# Autodesk Inventor assembly: 042-P(F,D-166-3)
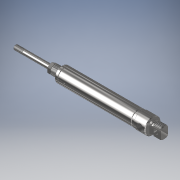
[picture p0: Inventor's stored thumbnail of the model, 180x180]
Saved by Autodesk Inventor 2017 (Build 210142000, 142)
## iProperties
Category: PARTsolutions
Company: BIMBA
Created: 2016-10-01
Part Number: 042-P(F,D-166-3)
Catalog Web Link: www.cadenas.de
Description: Original Line Standard Air Cylinders-
Vendor: BIMBA
Document SubType Name: Assembly
Designer: psAdmin
Manufacturer: BIMBA
PSOL_IDENT_0: {$CADENAS_DATA\23d-libs\bimba\bimba\bimba_imperial\bimba_full_line\original_line_cylinders\standard_
PSOL_IDENT_1: air_cylinders\standard_air_cylinder_asmtab.prj},321 {VTYP=3D},{STYP=ASSTAB},{NB=042-P(F,D-166-3)},{L
PSOL_IDENT_2: INA=042-P},{NN=Original Line Standard Air Cylinders},{DATE=22.09.2016 13:52:24},{GEOMDATE=11.07.2016
PSOL_IDENT_3: 10:37:18},{VERSION=},{LINEID=50},{LINESUBID=-1},{WBVAR=STROKE,ACTING,MNT,DER,NR,BM,CO,OO,VO,M,EE,EE
PSOL_IDENT_4: L,K,Q,Y,G,T,B,H,SER,SR,NT,W,HL,STPT1,STPT2,STPT3,STPT4,MB,PB,PRC,TB,MN}  {NB=042-P(F,D-166-3)},{LINA=
PSOL_IDENT_5: 042-P},{KT=DUMMY},{PN=042-P},{PNC=042-P(F,D-166-3)},{PNA=(D-166-3)},{DASH=-},{BORE1=0.75000000},{BOR
PSOL_IDENT_6: E=3/4\" (04)},{BOREPN=04},{STROKE=2.000},{STROKEALG=[0.011:50/0.001]},{STROKE1=2.000},{ACTING=},{ACT
PSOL_IDENT_7: INGALG= '' , 'Single Acting (SA)' , 'R' , 'Reverse Single Acting (SA)' , 'D' , 'Double Acting (SA)'
PSOL_IDENT_8: },{ACTINGPN=},{MNT=P},{MNTALG= '' , 'Front Nose Mounting (SA)' , 'P' , 'Rear Pivot Mounting (SA)' , '
PSOL_IDENT_9: BF' , 'Front Block Mounting (SA)' , 'BR' , 'Rear Block Mounting for Vertical Positioning (SA)' , 'BF
PSOL_IDENT_10: T' , 'Front Block Trunnion Mounting (SA)' , 'BRT' , 'Rear Block Trunnion Mounting (SA)' , 'A' , 'Dou
PSOL_IDENT_11: ble End Mounting with Brackets and Adjustable Stroke (SA)' , 'AP' , 'Rear Pivot Mounting with Adjust
PSOL_IDENT_12: able Stroke (SA)' },{TYPE=},{MNTPN=P},{DER=},{DERALG= '' , 'N/A' },{NR=},{NRALG= '' , 'Round (Standa
PSOL_IDENT_13: rd)' , 'NR' , 'Non-rotating - Hexagon Rod' },{NRPN=},{BM=},{BMALG= '' , 'N/A' },{BMPN=},{CO=},{COALG=
PSOL_IDENT_14: '' , 'N/A' },{OO=},{OOALG= '', 'N/A' },{OOPN=},{VO=Z},{VOALG= 'Z' , 'N/A' },{VOPN=},{OOVOPN=},{M=},
PSOL_IDENT_15: {MALG= '', 'Without Magnet', 'M', 'With Magnet' },{EE=},{EEL=0.000},{EEMAX=48.0000},{EEALG= '', 'Wit
PSOL_IDENT_16: hout Extra Extension', 'EE', 'With Extra Extension' },{EELALG=0},{EEPN=},{EEPN1=0.000},{K=},{KALG= ''
PSOL_IDENT_17: , 'Standard' , 'K' , 'Ports Rotated 90deg K' },{KPN=},{Q=},{QALG= '' , 'N/A' },{QPN=},{Y=},{YALG= ''
PSOL_IDENT_18: , 'Without Pivot Bushing' , 'Y' , 'With Pivot Bushing' },{YPN=},{YCON=},{F=},{FALG= '', 'Non-Coated
PSOL_IDENT_19: (Standard)', 'F', 'Molycoated' },{FPN=},{G=},{GPN=},{GPN99=},{T=},{TALG= '' , 'Standard -20° to 200
PSOL_IDENT_20: °F (-29° to 95°C)' , 'N' , 'Low Temperature' , 'V' , 'High Temperature' },{NPN=},{VPN=},{B=},{BALG= ''
PSOL_IDENT_21: , 'W/out Bumpers' , 'B' , 'W/ Bumpers' },{BPN=},{H=},{HALG= '', 'W/ Standard Spring (Relaxed 3 lbs./
PSOL_IDENT_22: Compressed 6 lbs.)', 'H', 'W/ Heavy Spring (Relaxed 4 lbs./Compressed 10 lbs.)' },{HPN=},{SER=},{SER
PSOL_IDENT_23: ALG= '' , 'N/A' },{SR=C},{SRALG= 'C' , 'Standard Blackened Carbon Steel' , 'SR' , 'Stainless Steel [
PSOL_IDENT_24: SR]' },{SRPN=},{SRCON=1},{NT=},{NTPN=},{W=},{WALG= '' , 'N/A' },{WPN=},{E=},{EALG= '' , 'Standard Se
PSOL_IDENT_25: als/Lube' , 'E' , 'Non-Lube Seals/Lube' },{EPN=},{HL=},{HLALG= '' , 'N/A' },{ST=},{STALG= '' , 'N/A'
PSOL_IDENT_26: },{STPT1=},{STPT1ALG= '' , 'N/A' },{STPT2=},{STPT2ALG= '' , 'N/A' },{STPT3=},{STPT3ALG= '' , 'N/A'
PSOL_IDENT_27: },{STPT4=},{STPT4ALG= '' , 'N/A' },{STPN=},{MB=},{MBALG= '' , 'N/A' },{MBPN=},{MBPNALL=},{MBPNALLREA
PSOL_IDENT_28: R=},{PB=},{PBALG= '' , 'Without Pivot Bracket' , 'D-167' , 'D-167' },{PBPN=},{PBPNALL=D-167},{PRC=F,
PSOL_IDENT_29: D-166-3},{PRCALG= '' , 'W/out Pivot Rod Clevis' , 'F,D-166-3' , 'D-166-3 (front)' },{PRCPN=(F,D-166-
PSOL_IDENT_30: 3)},{PRCPNALL=D-166-3},{TB=},{TBALG= '' , 'N/A' },{TBPN=},{TBPNALL=},{MN=},{MNALG= '' , 'Without Mou
PSOL_IDENT_31: nting Nut' , 'F,D-98' , 'D-98 (front)' , 'R,D-9' , 'D-9 (rear)', '2xZ' , 'D-98 (front) & D-9 (rear)'
PSOL_IDENT_32: },{MNPN=},{MNCONF=},{MNCONR=},{TLEN=3.9450},{FRAC=6.3500},{RGCON=},{RGDACCON=},{RHCON=P},{RHCON1=P}
PSOL_IDENT_33: ,{RHCONON=1},{RHACCON=},{FNUTCON=0},{RNUTCON=0},{FNUTPN=D-98},{RNUTPN=D-9},{FNUTTRANS=0.0000},{RNUTT
PSOL_IDENT_34: RANS=0.0000},{VHOLECON=2},{A1=0.8750},{A1N=0.8750},{A1P=1.5940},{A1B=1.5940},{A4=0.3130},{A4N=0.3130
PSOL_IDENT_35: },{A4P=0.2525},{A5=0.0300},{A1H=1.594},{A1NH=0.5310},{A1PH=1.5940},{A1BH=1.0940},{A1SH=1.2190},{A2H=
PSOL_IDENT_36: 0.2190},{A2NH=0.2190},{LENGTH=2.2800},{LENGTH1=2.2800},{LENGTH2=3.8100},{MUL=3.3800},{MUL11=3.3800},
PSOL_IDENT_37: {MUL22=5.38},{MUL33=3.3800},{MUL2=1.6900},{MUL211=1.6900},{MUL222=2.6900},{MUL233=1.6900},{SSS=4.000
PSOL_IDENT_38: 0},{RGLEN=0.5920},{RHLEN=1.1230},{SSS1=3.0000},{A13=1.3120},{DIF=0.0000},{G5=0.6250},{ON=0},{SSADD=0
PSOL_IDENT_39: .0000},{BADD=0.0000},{MADD=0.0000},{NVADD=0.0000},{TRACKL=3.6550},{TRACKCON=D-74168},{TRIMCON=0},{TR
PSOL_IDENT_40: IMCON1=0},{PINCON=D-51},{FSPACE=0.5311},{SPACE=0.0643},{TEXT=0.1125},{S1=1.0000},{D1=0.8050},{D1N=0.
PSOL_IDENT_41: 8050},{D1B=0.8625},{D1P=0.8325},{FA=0.750},{RA=0.0000},{PPATH=standard_air_cylinder_asmtpl.prj},{MAT
PSOL_IDENT_42: ALGHTML=<b>Standard Original Line:</b><dl><dt>Rod:</dt><dd>- Stainless Steel</dd><dd>&nbsp;&nbsp;(5/
PSOL_IDENT_43: 16 9/16 Bores)</dd><dd>- High Strength Carbon Steel</dd><dd>&nbsp;&nbsp;(3/4 3 Bore)</dd><dd>- Stain
PSOL_IDENT_44: less Steel</dd><dd>&nbsp;&nbsp;(X style DXP/DX/DXDE)</dd><dt>Bearings:</dt><dd>- Sintered Bronze</dd
PSOL_IDENT_45: ><dt>Body:</dt><dd>- 304 Stainless Steel</dd><dt>End Caps:</dt><dd>- Aluminum</dd><dt>Seals:</dt><dd
PSOL_IDENT_46: >- Buna N</dd></dl>},{ASSCFGPRA=04P},{MBPNA=},{MNPNA=},{PRCPNA=(D-166-3)},{ASSOPTACC=STPT4},{A=5.66}
PSOL_IDENT_47: ,{HADD=0.0000},{WFL=0.25},{QADD=0.000},{QADD1=0.440},{TEST=2.0000},{MNTB=},{STDNUTF=0},{STDNUTR=0},{
PSOL_IDENT_48: STRK2D=0},{X2D=2},{STROKESW=2.000},{EESW=0.000},{FCD=0},{BCD=0},{RCD=0},{CUSTADD=1.000},{FT=1/4-28 U
PSOL_IDENT_49: NF-2A},{FT1=1/4-28 UNF-2A},{FT2=5/8-18 UNF-2A},{PORT=1/8 NPT},{FT11=1/2-20 UNF-2A},{FT12=5/8-18 UNF-
PSOL_IDENT_50: 2A}
NN: Original Line Standard Air Cylinders
NT: Standard Male Thread
NB: 042-P(F,D-166-3)
NBSYN: $PNC.
LINA: 042-P
PN: 042-P
PNA: (D-166-3)
BORE: 3/4" [04]
STROKE: 2.000
ACTING: Standard Single
MNT: Rear Pivot [P]
DER: N/A
NR: Standard Round
BM: N/A
CO: N/A
OO: N/A
VO: N/A
M: Without Magnet Piston
EE: Standard Rod Extension
EEL: 0.000
K: Standard
Q: N/A
Y: Standard Pivot Style
G: Standard Grease Lube
T: Standard -20° to 200°F (-29° to 95°C)
B: Without Bumpers
H: Standard (3 - 6 lbs.)
SER: N/A
SR: Standard Blackened Carbon Steel
W: N/A
HL: N/A
STPT1: N/A
STPT2: N/A
STPT3: N/A
STPT4: N/A
MB: N/A
PB: Without Pivot Bracket
PRC: D-166-3 (front)
TB: N/A
MN: Without Mounting Nut
A: 5.66
SUPPLIER: BIMBA
ARTICLENO: 042-P(F,D-166-3)
BOMINFO: 042-P
CREATOR: CADENAS GmbH
Title: 042-P
Author: Cadenas PARTsolutions
## Documents named in this file (8)
- \\Mac\Home\Desktop\bunnybots 2016\15102898-16-Bunnybot-CAD\Bunnybot-To_be_renamed\15102898-16-A-0000\15102898-16-A-0200\Imported Components\Pistons\042-P(F,D-166-3).iam
- \\Mac\Home\Desktop\bunnybots 2016\15102898-16-Bunnybot-CAD\Bunnybot-To_be_renamed\15102898-16-A-0000\15102898-16-A-0200\Imported Components\Pistons\042-PC(F,D-166-3)0000_0_dummy.ipt
- \\Mac\Home\Desktop\bunnybots 2016\15102898-16-Bunnybot-CAD\Bunnybot-To_be_renamed\15102898-16-A-0000\15102898-16-A-0200\Imported Components\Pistons\04000-0_rod_guide.ipt
- \\Mac\Home\Desktop\bunnybots 2016\15102898-16-Bunnybot-CAD\Bunnybot-To_be_renamed\15102898-16-A-0000\15102898-16-A-0200\Imported Components\Pistons\04-3_9452C.ipt
- \\Mac\Home\Desktop\bunnybots 2016\15102898-16-Bunnybot-CAD\Bunnybot-To_be_renamed\15102898-16-A-0000\15102898-16-A-0200\Imported Components\Pistons\04P0000_rear_head.ipt
- \\Mac\Home\Desktop\bunnybots 2016\15102898-16-Bunnybot-CAD\Bunnybot-To_be_renamed\15102898-16-A-0000\15102898-16-A-0200\Imported Components\Pistons\C-042-P0_rod.ipt
- \\Mac\Home\Desktop\bunnybots 2016\15102898-16-Bunnybot-CAD\Bunnybot-To_be_renamed\15102898-16-A-0000\15102898-16-A-0200\Imported Components\Pistons\D-166-3-dummy.ipt
- \\Mac\Home\Desktop\bunnybots 2016\15102898-16-Bunnybot-CAD\Bunnybot-To_be_renamed\15102898-16-A-0000\15102898-16-A-0200\Imported Components\Pistons\D-344.ipt
## Components (7 placed, 7 different names)
1. 042-PC(F,D-166-3)0000_0_dummy:1
2. 04000-0_rod_guide:1
3. 04-3_9452C:1 — Mate:1
4. 04P0000_rear_head:1
5. C-042-P0_rod:1 — Mate:1
6. D-166-3-dummy:1
7. D-344:1
## Relationships (1: Mate 1)
- Mate:1: 04-3_9452C:1 ↔ C-042-P0_rod:1
